# Autodesk Inventor assembly: support orangepi
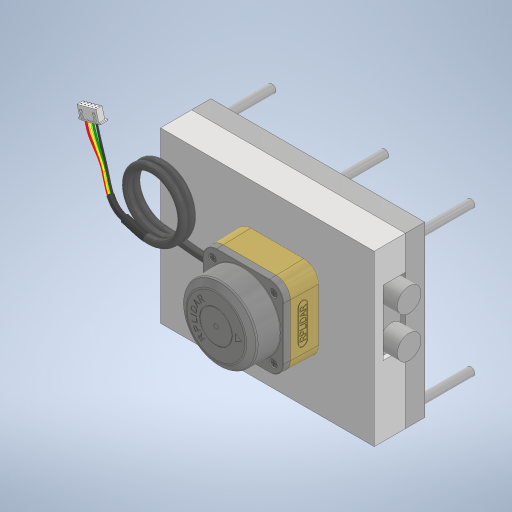
[picture p0: Inventor's stored thumbnail of the model, 512x512]
Saved by Autodesk Inventor 2024 (Build 280153000, 153)
## iProperties
Created: 2024-03-01
Part Number: support orangepi
Document SubType Name: Assembly
Designer: AdminForWorker
Title: support orangepi v17
Author: AdminForWorker
## Documents named in this file (12)
- C:\Users\phaly\Music\Perso\Projet voiture\3D\Support\support orangepi.iam
- C:\Users\phaly\Downloads\support orangepi v17\Component1.ipt
- C:\Users\phaly\Downloads\support orangepi v17\Component3.ipt
- C:\Users\phaly\Downloads\support orangepi v17\Component4.ipt
- C:\Users\phaly\Downloads\support orangepi v17\Component5.ipt
- C:\Users\phaly\Downloads\support orangepi v17\Component6.ipt
- C:\Users\phaly\Downloads\support orangepi v17\Component7.ipt
- C:\Users\phaly\Downloads\support orangepi v17\Component9.ipt
- C:\Users\phaly\Downloads\support orangepi v17\Component10.ipt
- C:\Users\phaly\Music\Perso\Projet voiture\3D\Support\support pile.ipt
- C:\Users\phaly\Music\Perso\Projet voiture\3D\Support\couvercle.ipt
- C:\Users\phaly\Music\Perso\Projet voiture\Documentation\LIDAR\3D\C1M1_appearance_V2_20230926.3d_model\C1M1_appearance_V2_20230926.3d_model.ipt
## Components (11 placed, 11 different names)
1. Component1:1 — Placage:7, Placage:8, Affleurement:1
2. Component3:1 — Placage:9, Affleurement:2, Placage:10
3. Component4:1 — Placage:11, Placage:12, Affleurement:3
4. Component5:1 — Placage:4, Placage:5, Placage:6
5. Component6:1 — Affleurement:4, Placage:13, Placage:14
6. Component7:1 — Placage:4, Placage:5, Placage:6, Placage:7, Placage:8, Affleurement:1, Placage:9, Affleurement:2, Placage:10, Placage:11, Placage:12, Affleurement:3, Affleurement:4, Placage:13, Placage:14, Placage:15, Placage:16, Placage:17, Placage:18
7. Component9:1
8. Component10:1
9. support pile:1 — Placage:15, Placage:16, Placage:17
10. couvercle:1 — Placage:18, Placage:19
11. C1M1_appearance_V2_20230926.3d_model:1 — Placage:19
## Relationships (20: Mate 16, Flush 4)
- Placage:4 [Mate]: Component5:1 ↔ Component7:1
- Placage:5 [Mate]: Component5:1 ↔ Component7:1
- Placage:6 [Mate]: Component5:1 ↔ Component7:1
- Placage:7 [Mate]: Component1:1 ↔ Component7:1
- Placage:8 [Mate]: Component1:1 ↔ Component7:1
- Affleurement:1 [Flush]: Component1:1 ↔ Component7:1
- Placage:9 [Mate]: Component3:1 ↔ Component7:1
- Affleurement:2 [Flush]: Component3:1 ↔ Component7:1
- Placage:10 [Mate]: Component3:1 ↔ Component7:1
- Placage:11 [Mate]: Component4:1 ↔ Component7:1
- Placage:12 [Mate]: Component4:1 ↔ Component7:1
- Affleurement:3 [Flush]: Component4:1 ↔ Component7:1
- Affleurement:4 [Flush]: Component6:1 ↔ Component7:1
- Placage:13 [Mate]: Component6:1 ↔ Component7:1
- Placage:14 [Mate]: Component6:1 ↔ Component7:1
- Placage:15 [Mate]: Component7:1 ↔ support pile:1
- Placage:16 [Mate]: Component7:1 ↔ support pile:1
- Placage:17 [Mate]: Component7:1 ↔ support pile:1
- Placage:18 [Mate]: Component7:1 ↔ couvercle:1
- Placage:19 [Mate]: couvercle:1 ↔ C1M1_appearance_V2_20230926.3d_model:1
